# Autodesk Inventor assembly: Osnova
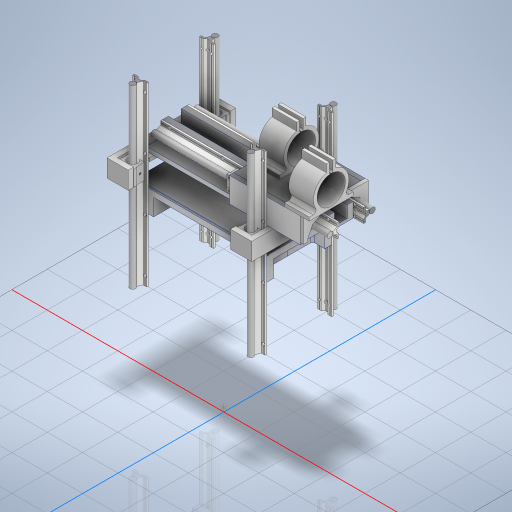
[picture p0: Inventor's stored thumbnail of the model, 512x512]
Saved by Autodesk Inventor 2024 (Build 280153000, 153)
## iProperties
Created: 2023-08-21
Part Number: Osnova
Document SubType Name: Assembly
Designer: KirikDK
Mass: 35023.4 g
Surface Area: 34965 cm^2
Volume: 16941.4 cm^3
Density: 2.06732 g/cm^3
Author: KirikDK
## Documents named in this file (12)
- C:\WorkProject\CNC_Lathe\MiniTocatka\Support.iam
- C:\WorkProject\CNC_Lathe\MiniTocatka\Bear.ipt
- C:\WorkProject\CNC_Lathe\MiniTocatka\PlasticZasita.ipt
- C:\WorkProject\CNC_Lathe\MiniTocatka\sbr16 (ap242)\0_8.ipt
- C:\WorkProject\CNC_Lathe\MiniTocatka\Y_karetka_A.ipt
- C:\WorkProject\CNC_Lathe\MiniTocatka\Y_karetka_B.ipt
- C:\WorkProject\CNC_Lathe\MiniTocatka\MainRails300_A.ipt
- C:\WorkProject\CNC_Lathe\MiniTocatka\MainRails300_B.ipt
- C:\WorkProject\CNC_Lathe\MiniTocatka\FlanecElement.ipt
- C:\WorkProject\CNC_Lathe\MiniTocatka\ZadBabkaOsnova.ipt
- C:\WorkProject\CNC_Lathe\MiniTocatka\VerticalAxis.ipt
- C:\WorkProject\CNC_Lathe\MiniTocatka\MotorClampMain.ipt
## Components (23 placed, 11 different names)
1. PlasticZasita:1
2. Y_karetka_A:1 — Mate:250, Mate:251, Flush:111, Mate:263, Mate:276, Flush:134, Flush:135, Flush:137, Flush:138
3. Y_karetka_B:1 — Mate:250, Mate:251, Flush:111, Mate:262, Mate:278, Mate:279
4. MainRails300_A:1 — Mate:252, Mate:253, Flush:112, Mate:254, Mate:256, Flush:114, Mate:262
5. MainRails300_B:1 — Mate:252, Mate:253, Flush:112, Mate:255, Mate:257, Flush:113, Mate:259, Mate:261, Mate:275, Flush:136, Mate:277
6. 0_8:6 — Mate:254, Mate:255, Flush:113, Mate:260
7. 0_8:7 — Mate:256, Mate:257, Flush:114, Mate:258
8. Bear:31 — Mate:258, Mate:259, Mate:263
9. Bear:32 — Mate:260, Mate:261
10. ZadBabkaOsnova:1 — Mate:265, Flush:117, Flush:118, Mate:266, Flush:119, Flush:120, Mate:267, Flush:121, Flush:122, Mate:268, Flush:123, Flush:124
11. 0_8:11 — Mate:266, Flush:119, Flush:120, Mate:271, Mate:277
12. 0_8:12 — Mate:265, Flush:117, Flush:118, Mate:270
13. 0_8:14 — Mate:268, Flush:123, Flush:124, Mate:269
14. 0_8:15 — Mate:267, Flush:121, Flush:122, Mate:272
15. Bear:33 — Mate:269, Flush:125, Flush:126, Flush:131
16. Bear:34 — Mate:270, Flush:125, Flush:126
17. Bear:35 — Mate:271, Flush:127, Flush:128, Mate:274, Flush:132, Flush:133
18. Bear:36 — Mate:272, Flush:127, Flush:128, Mate:273, Flush:129, Flush:130, Flush:131
19. VerticalAxis:1 — Mate:273, Flush:129, Flush:130, Mate:275, Flush:136
20. VerticalAxis:2 — Mate:274, Flush:132, Flush:133
21. FlanecElement:2 — Mate:276, Flush:134, Flush:135
22. MotorClampMain:2 — Mate:279, Flush:138
23. MotorClampMain:3 — Mate:278, Flush:137
## Relationships (55: Mate 29, Flush 26)
- Mate:250: Y_karetka_A:1 ↔ Y_karetka_B:1
- Mate:251: Y_karetka_A:1 ↔ Y_karetka_B:1
- Flush:111: Y_karetka_A:1 ↔ Y_karetka_B:1
- Mate:252: MainRails300_A:1 ↔ MainRails300_B:1
- Mate:253: MainRails300_A:1 ↔ MainRails300_B:1
- Flush:112: MainRails300_A:1 ↔ MainRails300_B:1
- Mate:254: MainRails300_A:1 ↔ 0_8:6
- Mate:255: MainRails300_B:1 ↔ 0_8:6
- Mate:256: MainRails300_A:1 ↔ 0_8:7
- Mate:257: MainRails300_B:1 ↔ 0_8:7
- Flush:113: MainRails300_B:1 ↔ 0_8:6
- Flush:114: MainRails300_A:1 ↔ 0_8:7
- Mate:258: 0_8:7 ↔ Bear:31
- Mate:259: MainRails300_B:1 ↔ Bear:31
- Mate:260: 0_8:6 ↔ Bear:32
- Mate:261: MainRails300_B:1 ↔ Bear:32
- Mate:262: Y_karetka_B:1 ↔ MainRails300_A:1
- Mate:263: Y_karetka_A:1 ↔ Bear:31
- Mate:265: ZadBabkaOsnova:1 ↔ 0_8:12
- Flush:117: ZadBabkaOsnova:1 ↔ 0_8:12
- Flush:118: ZadBabkaOsnova:1 ↔ 0_8:12
- Mate:266: ZadBabkaOsnova:1 ↔ 0_8:11
- Flush:119: ZadBabkaOsnova:1 ↔ 0_8:11
- Flush:120: ZadBabkaOsnova:1 ↔ 0_8:11
- Mate:267: ZadBabkaOsnova:1 ↔ 0_8:15
- Flush:121: ZadBabkaOsnova:1 ↔ 0_8:15
- Flush:122: ZadBabkaOsnova:1 ↔ 0_8:15
- Mate:268: ZadBabkaOsnova:1 ↔ 0_8:14
- Flush:123: ZadBabkaOsnova:1 ↔ 0_8:14
- Flush:124: ZadBabkaOsnova:1 ↔ 0_8:14
- Mate:269: 0_8:14 ↔ Bear:33
- Mate:270: 0_8:12 ↔ Bear:34
- Flush:125: Bear:33 ↔ Bear:34
- Flush:126: Bear:33 ↔ Bear:34
- Mate:271: 0_8:11 ↔ Bear:35
- Mate:272: 0_8:15 ↔ Bear:36
- Flush:127: Bear:35 ↔ Bear:36
- Flush:128: Bear:35 ↔ Bear:36
- Mate:273: Bear:36 ↔ VerticalAxis:1
- Flush:129: Bear:36 ↔ VerticalAxis:1
- Flush:130: Bear:36 ↔ VerticalAxis:1
- Flush:131: Bear:33 ↔ Bear:36
- Mate:274: Bear:35 ↔ VerticalAxis:2
- Flush:132: Bear:35 ↔ VerticalAxis:2
- Flush:133: Bear:35 ↔ VerticalAxis:2
- Mate:275: MainRails300_B:1 ↔ VerticalAxis:1
- Mate:276: Y_karetka_A:1 ↔ FlanecElement:2
- Flush:134: Y_karetka_A:1 ↔ FlanecElement:2
- Flush:135: Y_karetka_A:1 ↔ FlanecElement:2
- Flush:136: MainRails300_B:1 ↔ VerticalAxis:1
- Mate:277 (12 mm): MainRails300_B:1 ↔ 0_8:11
- Mate:278: Y_karetka_B:1 ↔ MotorClampMain:3
- Mate:279: Y_karetka_B:1 ↔ MotorClampMain:2
- Flush:137: Y_karetka_A:1 ↔ MotorClampMain:3
- Flush:138: Y_karetka_A:1 ↔ MotorClampMain:2
